# Autodesk Inventor assembly: slider
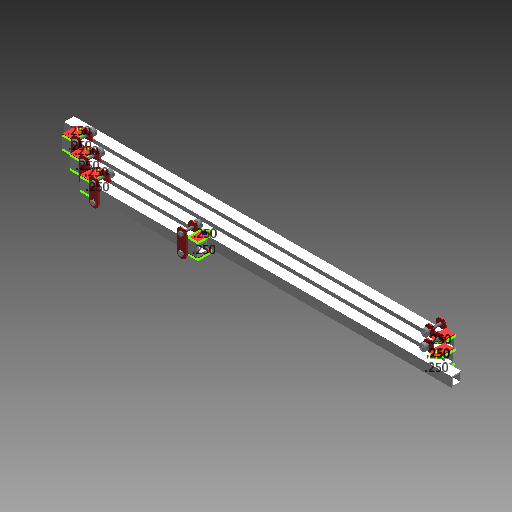
[picture p0: Inventor's stored thumbnail of the model, 512x512]
Saved by Autodesk Inventor 2019 (Build 230136000, 136)
## iProperties
Created: 2019-01-13
Part Number: slider
Document SubType Name: Assembly
Designer: lebraddock
Mass: 2872.54 g
Surface Area: 7390.42 cm^2
Volume: 1092.69 cm^3
Density: 2.62887 g/cm^3
Author: lebraddock
## Documents named in this file (9)
- C:\Users\lebraddock\Documents\CameronsRoboticsThings\2019 CAD\slider.iam
- C:\Users\lebraddock\Documents\CameronsRoboticsThings\2019 CAD\41inch 1x1 liftfirstbar.ipt
- C:\Users\lebraddock\Documents\CameronsRoboticsThings\2019 CAD\linear_slide_piece2_v2.ipt
- C:\Users\lebraddock\Documents\CameronsRoboticsThings\2019 CAD\linearSlide_piece1_v2.ipt
- C:\Users\lebraddock\Documents\CameronsRoboticsThings\2019 CAD\1x1 plate spacer.ipt
- C:\Users\lebraddock\Documents\CameronsRoboticsThings\2019 CAD\spacerslide.ipt
- C:\Users\lebraddock\Documents\CameronsRoboticsThings\2019 CAD\93306A555_ALUMINUM HEX HEAD CAP SCREW.ipt
- C:\Users\lebraddock\Documents\CameronsRoboticsThings\2019 CAD\60355K440_BALL BEARING.ipt
- C:\Users\lebraddock\Documents\CameronsRoboticsThings\2019 CAD\12sliderbar.ipt
## Components (70 placed, 8 different names)
1. 41inch 1x1 liftfirstbar:1 — Mate:1, Flush:1, Flush:2, Mate:2, Flush:3, Flush:4, Mate:3, Flush:5, Flush:6, Mate:4, Flush:7, Flush:8, Mate:5, Flush:9, Tangent:1, Mate:6, Flush:10, Tangent:2, Tangent:5, Tangent:7
2. linear_slide_piece2_v2:1 — Mate:6, Flush:10, Tangent:2, Mate:27, Mate:29
3. linearSlide_piece1_v2:1 — Mate:4, Flush:7, Flush:8, Mate:14
4. linear_slide_piece2_v2:2 — Mate:5, Flush:9, Tangent:1, Mate:19, Mate:20, Mate:21, Mate:22
5. linearSlide_piece1_v2:2 — Mate:1, Flush:1, Flush:2, Insert:2
6. 1x1 plate spacer:1 — Mate:3, Flush:5, Flush:6
7. 1x1 plate spacer:2 — Mate:2, Flush:3, Flush:4
8. spacerslide:2 — Mate:14, Insert:2, Tangent:6
9. 93306A555_ALUMINUM HEX HEAD CAP SCREW:1 — Mate:19, Mate:20, Mate:30
10. 93306A555_ALUMINUM HEX HEAD CAP SCREW:2 — Mate:21, Mate:22, Mate:28
11. 60355K440_BALL BEARING:1 — Mate:29, Mate:30, Tangent:8
12. 60355K440_BALL BEARING:2 — Mate:27, Mate:28
13. 12sliderbar:1 — Mate:99, Flush:53, Flush:54, Flush:55, Flush:56, Mate:101, Flush:57, Flush:58, Flush:59, Flush:60, Mate:103, Flush:61, Mate:104, Flush:62, Tangent:21, Tangent:22, Mate:105, Flush:63, Flush:64, Mate:106, Flush:65, Flush:66, Flush:68, Flush:69, Flush:70, Mate:110, Flush:71, Tangent:24, Mate:111, Flush:72, Tangent:25
14. 41inch 1x1 liftfirstbar:2 — Tangent:6, Tangent:8, Mate:68, Flush:31, Flush:32, Flush:33, Flush:34, Flush:35, Flush:36, Flush:37, Flush:38, Mate:70, Flush:39, Flush:40, Mate:72, Flush:41, Tangent:11, Mate:73, Flush:42, Tangent:17, Tangent:19
15. linear_slide_piece2_v2:3
16. linearSlide_piece1_v2:3
17. linear_slide_piece2_v2:4
18. linearSlide_piece1_v2:4
19. 1x1 plate spacer:3
20. 1x1 plate spacer:4
21. spacerslide:3 — Tangent:5
22. 93306A555_ALUMINUM HEX HEAD CAP SCREW:3
23. 93306A555_ALUMINUM HEX HEAD CAP SCREW:4
24. 60355K440_BALL BEARING:3 — Tangent:7
25. 60355K440_BALL BEARING:4
26. linear_slide_piece2_v2:7 — Mate:73, Flush:42
27. linearSlide_piece1_v2:7 — Mate:69, Flush:32, Flush:33, Flush:36, Mate:89
28. linear_slide_piece2_v2:8 — Mate:72, Flush:41
29. linearSlide_piece1_v2:8 — Mate:71, Flush:39, Flush:40, Tangent:15
30. 1x1 plate spacer:7 — Mate:68, Flush:31, Mate:69, Flush:34, Flush:35
31. 1x1 plate spacer:8 — Flush:37, Flush:38, Mate:70, Mate:71
32. 93306A555_ALUMINUM HEX HEAD CAP SCREW:7 — Tangent:11
33. 93306A555_ALUMINUM HEX HEAD CAP SCREW:8
34. 60355K440_BALL BEARING:7 — Tangent:16
35. 60355K440_BALL BEARING:8
36. 41inch 1x1 liftfirstbar:3 — Tangent:16, Tangent:18, Tangent:31, Tangent:32, Tangent:33, Tangent:34
37. linear_slide_piece2_v2:9
38. linearSlide_piece1_v2:9 — Mate:88
39. linear_slide_piece2_v2:10
40. linearSlide_piece1_v2:10 — Tangent:14
41. 1x1 plate spacer:9
42. 1x1 plate spacer:10
43. 93306A555_ALUMINUM HEX HEAD CAP SCREW:9
44. 93306A555_ALUMINUM HEX HEAD CAP SCREW:10
45. 60355K440_BALL BEARING:9 — Tangent:17
46. 60355K440_BALL BEARING:10
47. spacerslide:4 — Mate:89, Tangent:15, Tangent:18
48. spacerslide:5 — Mate:88, Tangent:14, Tangent:19
49. linear_slide_piece2_v2:11 — Mate:104, Flush:62, Tangent:22
50. linearSlide_piece1_v2:11 — Mate:102, Flush:59, Flush:60
51. linear_slide_piece2_v2:12 — Mate:103, Flush:61
52. linearSlide_piece1_v2:12 — Mate:100, Flush:55, Flush:56
53. 1x1 plate spacer:11 — Mate:101, Flush:57, Flush:58, Mate:102
54. 1x1 plate spacer:12 — Mate:99, Flush:53, Flush:54, Mate:100
55. 93306A555_ALUMINUM HEX HEAD CAP SCREW:11 — Tangent:21
56. 93306A555_ALUMINUM HEX HEAD CAP SCREW:12
57. 60355K440_BALL BEARING:11 — Tangent:31
58. 60355K440_BALL BEARING:12
59. spacerslide:6 — Tangent:33
60. linear_slide_piece2_v2:13 — Mate:110, Flush:71, Tangent:24, Mate:112, Mate:113
61. linearSlide_piece1_v2:13 — Mate:107, Flush:67, Flush:68, Mate:109
62. linear_slide_piece2_v2:14 — Mate:111, Flush:72, Tangent:25, Tangent:26, Mate:114, Tangent:29, Mate:115
63. linearSlide_piece1_v2:14 — Mate:108, Flush:69, Flush:70, Tangent:23
64. 1x1 plate spacer:13 — Mate:105, Flush:63, Flush:64, Mate:107, Flush:67
65. 1x1 plate spacer:14 — Mate:106, Flush:65, Flush:66, Mate:108
66. 60355K440_BALL BEARING:13 — Mate:115, Tangent:30
67. 60355K440_BALL BEARING:14 — Mate:114, Tangent:28, Tangent:32
68. spacerslide:7 — Mate:109, Tangent:23, Tangent:34
69. 93306A555_ALUMINUM HEX HEAD CAP SCREW:13 — Mate:112, Tangent:26, Tangent:28
70. 93306A555_ALUMINUM HEX HEAD CAP SCREW:14 — Mate:113, Tangent:29, Tangent:30
## Relationships (181: Mate 86, Flush 62, Tangent 31, Insert 2)
- Mate:1 (3.175 mm): 41inch 1x1 liftfirstbar:1 ↔ linearSlide_piece1_v2:2
- Flush:1: 41inch 1x1 liftfirstbar:1 ↔ linearSlide_piece1_v2:2
- Flush:2: 41inch 1x1 liftfirstbar:1 ↔ linearSlide_piece1_v2:2
- Mate:2: 41inch 1x1 liftfirstbar:1 ↔ 1x1 plate spacer:2
- Flush:3: 41inch 1x1 liftfirstbar:1 ↔ 1x1 plate spacer:2
- Flush:4: 41inch 1x1 liftfirstbar:1 ↔ 1x1 plate spacer:2
- Mate:3: 41inch 1x1 liftfirstbar:1 ↔ 1x1 plate spacer:1
- Flush:5: 41inch 1x1 liftfirstbar:1 ↔ 1x1 plate spacer:1
- Flush:6: 41inch 1x1 liftfirstbar:1 ↔ 1x1 plate spacer:1
- Mate:4 (3.175 mm): 41inch 1x1 liftfirstbar:1 ↔ linearSlide_piece1_v2:1
- Flush:7: 41inch 1x1 liftfirstbar:1 ↔ linearSlide_piece1_v2:1
- Flush:8: 41inch 1x1 liftfirstbar:1 ↔ linearSlide_piece1_v2:1
- Mate:5: 41inch 1x1 liftfirstbar:1 ↔ linear_slide_piece2_v2:2
- Flush:9 (25.4 mm): 41inch 1x1 liftfirstbar:1 ↔ linear_slide_piece2_v2:2
- Tangent:1 (6.35 mm): 41inch 1x1 liftfirstbar:1 ↔ linear_slide_piece2_v2:2
- Mate:6: 41inch 1x1 liftfirstbar:1 ↔ linear_slide_piece2_v2:1
- Flush:10 (25.4 mm): 41inch 1x1 liftfirstbar:1 ↔ linear_slide_piece2_v2:1
- Tangent:2 (6.35 mm): 41inch 1x1 liftfirstbar:1 ↔ linear_slide_piece2_v2:1
- Mate:14: linearSlide_piece1_v2:1 ↔ spacerslide:2
- Insert:2: linearSlide_piece1_v2:2 ↔ spacerslide:2
- Mate:19: linear_slide_piece2_v2:2 ↔ 93306A555_ALUMINUM HEX HEAD CAP SCREW:1
- Mate:20: linear_slide_piece2_v2:2 ↔ 93306A555_ALUMINUM HEX HEAD CAP SCREW:1
- Mate:21: linear_slide_piece2_v2:2 ↔ 93306A555_ALUMINUM HEX HEAD CAP SCREW:2
- Mate:22: linear_slide_piece2_v2:2 ↔ 93306A555_ALUMINUM HEX HEAD CAP SCREW:2
- Mate:27 (7.112 mm): linear_slide_piece2_v2:1 ↔ 60355K440_BALL BEARING:2
- Mate:28: 93306A555_ALUMINUM HEX HEAD CAP SCREW:2 ↔ 60355K440_BALL BEARING:2
- Mate:29 (7.112 mm): linear_slide_piece2_v2:1 ↔ 60355K440_BALL BEARING:1
- Mate:30: 93306A555_ALUMINUM HEX HEAD CAP SCREW:1 ↔ 60355K440_BALL BEARING:1
- [Mate] (3.175 mm): 41inch 1x1 liftfirstbar:2 ↔ linearSlide_piece1_v2:4
- [Flush]: 41inch 1x1 liftfirstbar:2 ↔ linearSlide_piece1_v2:4
- [Flush]: 41inch 1x1 liftfirstbar:2 ↔ linearSlide_piece1_v2:4
- [Mate]: 41inch 1x1 liftfirstbar:2 ↔ 1x1 plate spacer:4
- [Flush]: 41inch 1x1 liftfirstbar:2 ↔ 1x1 plate spacer:4
- [Flush]: 41inch 1x1 liftfirstbar:2 ↔ 1x1 plate spacer:4
- [Mate]: 41inch 1x1 liftfirstbar:2 ↔ 1x1 plate spacer:3
- [Flush]: 41inch 1x1 liftfirstbar:2 ↔ 1x1 plate spacer:3
- [Flush]: 41inch 1x1 liftfirstbar:2 ↔ 1x1 plate spacer:3
- [Mate] (3.175 mm): 41inch 1x1 liftfirstbar:2 ↔ linearSlide_piece1_v2:3
- [Flush]: 41inch 1x1 liftfirstbar:2 ↔ linearSlide_piece1_v2:3
- [Flush]: 41inch 1x1 liftfirstbar:2 ↔ linearSlide_piece1_v2:3
- [Mate]: 41inch 1x1 liftfirstbar:2 ↔ linear_slide_piece2_v2:4
- [Flush] (25.4 mm): 41inch 1x1 liftfirstbar:2 ↔ linear_slide_piece2_v2:4
- [Tangent] (6.35 mm): 41inch 1x1 liftfirstbar:2 ↔ linear_slide_piece2_v2:4
- [Mate]: 41inch 1x1 liftfirstbar:2 ↔ linear_slide_piece2_v2:3
- [Flush] (25.4 mm): 41inch 1x1 liftfirstbar:2 ↔ linear_slide_piece2_v2:3
- [Tangent] (6.35 mm): 41inch 1x1 liftfirstbar:2 ↔ linear_slide_piece2_v2:3
- [Mate]: linearSlide_piece1_v2:3 ↔ spacerslide:3
- [Insert]: linearSlide_piece1_v2:4 ↔ spacerslide:3
- [Mate]: linear_slide_piece2_v2:4 ↔ 93306A555_ALUMINUM HEX HEAD CAP SCREW:3
- [Mate]: linear_slide_piece2_v2:4 ↔ 93306A555_ALUMINUM HEX HEAD CAP SCREW:3
- [Mate]: linear_slide_piece2_v2:4 ↔ 93306A555_ALUMINUM HEX HEAD CAP SCREW:4
- [Mate]: linear_slide_piece2_v2:4 ↔ 93306A555_ALUMINUM HEX HEAD CAP SCREW:4
- [Mate] (7.112 mm): linear_slide_piece2_v2:3 ↔ 60355K440_BALL BEARING:4
- [Mate]: 93306A555_ALUMINUM HEX HEAD CAP SCREW:4 ↔ 60355K440_BALL BEARING:4
- [Mate] (7.112 mm): linear_slide_piece2_v2:3 ↔ 60355K440_BALL BEARING:3
- [Mate]: 93306A555_ALUMINUM HEX HEAD CAP SCREW:3 ↔ 60355K440_BALL BEARING:3
- Tangent:5: 41inch 1x1 liftfirstbar:1 ↔ spacerslide:3
- Tangent:6: spacerslide:2 ↔ 41inch 1x1 liftfirstbar:2
- Tangent:7: 41inch 1x1 liftfirstbar:1 ↔ 60355K440_BALL BEARING:3
- Tangent:8: 60355K440_BALL BEARING:1 ↔ 41inch 1x1 liftfirstbar:2
- [Mate]: linear_slide_piece2_v2:8 ↔ 93306A555_ALUMINUM HEX HEAD CAP SCREW:7
- [Mate]: linear_slide_piece2_v2:8 ↔ 93306A555_ALUMINUM HEX HEAD CAP SCREW:7
- [Mate]: linear_slide_piece2_v2:8 ↔ 93306A555_ALUMINUM HEX HEAD CAP SCREW:8
- [Mate]: linear_slide_piece2_v2:8 ↔ 93306A555_ALUMINUM HEX HEAD CAP SCREW:8
- [Mate] (7.112 mm): linear_slide_piece2_v2:7 ↔ 60355K440_BALL BEARING:8
- [Mate]: 93306A555_ALUMINUM HEX HEAD CAP SCREW:8 ↔ 60355K440_BALL BEARING:8
- [Mate] (7.112 mm): linear_slide_piece2_v2:7 ↔ 60355K440_BALL BEARING:7
- [Mate]: 93306A555_ALUMINUM HEX HEAD CAP SCREW:7 ↔ 60355K440_BALL BEARING:7
- Mate:68: 41inch 1x1 liftfirstbar:2 ↔ 1x1 plate spacer:7
- Flush:31: 41inch 1x1 liftfirstbar:2 ↔ 1x1 plate spacer:7
- Mate:69: linearSlide_piece1_v2:7 ↔ 1x1 plate spacer:7
- Flush:32: 41inch 1x1 liftfirstbar:2 ↔ linearSlide_piece1_v2:7
- Flush:33: 41inch 1x1 liftfirstbar:2 ↔ linearSlide_piece1_v2:7
- Flush:34: 41inch 1x1 liftfirstbar:2 ↔ 1x1 plate spacer:7
- Flush:35: 41inch 1x1 liftfirstbar:2 ↔ 1x1 plate spacer:7
- Flush:36: 41inch 1x1 liftfirstbar:2 ↔ linearSlide_piece1_v2:7
- Flush:37: 41inch 1x1 liftfirstbar:2 ↔ 1x1 plate spacer:8
- Flush:38: 41inch 1x1 liftfirstbar:2 ↔ 1x1 plate spacer:8
- Mate:70: 41inch 1x1 liftfirstbar:2 ↔ 1x1 plate spacer:8
- Mate:71: linearSlide_piece1_v2:8 ↔ 1x1 plate spacer:8
- Flush:39: 41inch 1x1 liftfirstbar:2 ↔ linearSlide_piece1_v2:8
- Flush:40: 41inch 1x1 liftfirstbar:2 ↔ linearSlide_piece1_v2:8
- Mate:72: 41inch 1x1 liftfirstbar:2 ↔ linear_slide_piece2_v2:8
- Flush:41 (25.4 mm): 41inch 1x1 liftfirstbar:2 ↔ linear_slide_piece2_v2:8
- Tangent:11 (6.35 mm): 41inch 1x1 liftfirstbar:2 ↔ 93306A555_ALUMINUM HEX HEAD CAP SCREW:7
- Mate:73: 41inch 1x1 liftfirstbar:2 ↔ linear_slide_piece2_v2:7
- Flush:42 (25.4 mm): 41inch 1x1 liftfirstbar:2 ↔ linear_slide_piece2_v2:7
- [Mate] (3.175 mm): 41inch 1x1 liftfirstbar:3 ↔ linearSlide_piece1_v2:10
- [Flush]: 41inch 1x1 liftfirstbar:3 ↔ linearSlide_piece1_v2:10
- [Flush]: 41inch 1x1 liftfirstbar:3 ↔ linearSlide_piece1_v2:10
- [Mate]: 41inch 1x1 liftfirstbar:3 ↔ 1x1 plate spacer:10
- [Flush]: 41inch 1x1 liftfirstbar:3 ↔ 1x1 plate spacer:10
- [Flush]: 41inch 1x1 liftfirstbar:3 ↔ 1x1 plate spacer:10
- [Mate]: 41inch 1x1 liftfirstbar:3 ↔ 1x1 plate spacer:9
- [Flush]: 41inch 1x1 liftfirstbar:3 ↔ 1x1 plate spacer:9
- [Flush]: 41inch 1x1 liftfirstbar:3 ↔ 1x1 plate spacer:9
- [Mate] (3.175 mm): 41inch 1x1 liftfirstbar:3 ↔ linearSlide_piece1_v2:9
- [Flush]: 41inch 1x1 liftfirstbar:3 ↔ linearSlide_piece1_v2:9
- [Flush]: 41inch 1x1 liftfirstbar:3 ↔ linearSlide_piece1_v2:9
- [Mate]: 41inch 1x1 liftfirstbar:3 ↔ linear_slide_piece2_v2:10
- [Flush] (25.4 mm): 41inch 1x1 liftfirstbar:3 ↔ linear_slide_piece2_v2:10
- [Tangent] (6.35 mm): 41inch 1x1 liftfirstbar:3 ↔ linear_slide_piece2_v2:10
- [Mate]: 41inch 1x1 liftfirstbar:3 ↔ linear_slide_piece2_v2:9
- [Flush] (25.4 mm): 41inch 1x1 liftfirstbar:3 ↔ linear_slide_piece2_v2:9
- [Tangent] (6.35 mm): 41inch 1x1 liftfirstbar:3 ↔ linear_slide_piece2_v2:9
- [Mate]: linear_slide_piece2_v2:10 ↔ 93306A555_ALUMINUM HEX HEAD CAP SCREW:9
- [Mate]: linear_slide_piece2_v2:10 ↔ 93306A555_ALUMINUM HEX HEAD CAP SCREW:9
- [Mate]: linear_slide_piece2_v2:10 ↔ 93306A555_ALUMINUM HEX HEAD CAP SCREW:10
- [Mate]: linear_slide_piece2_v2:10 ↔ 93306A555_ALUMINUM HEX HEAD CAP SCREW:10
- [Mate] (7.112 mm): linear_slide_piece2_v2:9 ↔ 60355K440_BALL BEARING:10
- [Mate]: 93306A555_ALUMINUM HEX HEAD CAP SCREW:10 ↔ 60355K440_BALL BEARING:10
- [Mate] (7.112 mm): linear_slide_piece2_v2:9 ↔ 60355K440_BALL BEARING:9
- [Mate]: 93306A555_ALUMINUM HEX HEAD CAP SCREW:9 ↔ 60355K440_BALL BEARING:9
- Mate:88: linearSlide_piece1_v2:9 ↔ spacerslide:5
- Tangent:14: linearSlide_piece1_v2:10 ↔ spacerslide:5
- Mate:89: linearSlide_piece1_v2:7 ↔ spacerslide:4
- Tangent:15: linearSlide_piece1_v2:8 ↔ spacerslide:4
- Tangent:16: 60355K440_BALL BEARING:7 ↔ 41inch 1x1 liftfirstbar:3
- Tangent:17: 41inch 1x1 liftfirstbar:2 ↔ 60355K440_BALL BEARING:9
- Tangent:18: 41inch 1x1 liftfirstbar:3 ↔ spacerslide:4
- Tangent:19: 41inch 1x1 liftfirstbar:2 ↔ spacerslide:5
- [Mate]: linear_slide_piece2_v2:12 ↔ 93306A555_ALUMINUM HEX HEAD CAP SCREW:11
- [Mate]: linear_slide_piece2_v2:12 ↔ 93306A555_ALUMINUM HEX HEAD CAP SCREW:11
- [Mate]: linear_slide_piece2_v2:12 ↔ 93306A555_ALUMINUM HEX HEAD CAP SCREW:12
- [Mate]: linear_slide_piece2_v2:12 ↔ 93306A555_ALUMINUM HEX HEAD CAP SCREW:12
- [Mate] (7.112 mm): linear_slide_piece2_v2:11 ↔ 60355K440_BALL BEARING:12
- [Mate]: 93306A555_ALUMINUM HEX HEAD CAP SCREW:12 ↔ 60355K440_BALL BEARING:12
- [Mate] (7.112 mm): linear_slide_piece2_v2:11 ↔ 60355K440_BALL BEARING:11
- [Mate]: 93306A555_ALUMINUM HEX HEAD CAP SCREW:11 ↔ 60355K440_BALL BEARING:11
- [Mate]: linearSlide_piece1_v2:11 ↔ spacerslide:6
- [Tangent]: linearSlide_piece1_v2:12 ↔ spacerslide:6
- Mate:99: 12sliderbar:1 ↔ 1x1 plate spacer:12
- Flush:53: 12sliderbar:1 ↔ 1x1 plate spacer:12
- Flush:54: 12sliderbar:1 ↔ 1x1 plate spacer:12
- Mate:100: linearSlide_piece1_v2:12 ↔ 1x1 plate spacer:12
- Flush:55: 12sliderbar:1 ↔ linearSlide_piece1_v2:12
- Flush:56: 12sliderbar:1 ↔ linearSlide_piece1_v2:12
- Mate:101: 12sliderbar:1 ↔ 1x1 plate spacer:11
- Flush:57: 12sliderbar:1 ↔ 1x1 plate spacer:11
- Flush:58: 12sliderbar:1 ↔ 1x1 plate spacer:11
- Mate:102: linearSlide_piece1_v2:11 ↔ 1x1 plate spacer:11
- Flush:59: 12sliderbar:1 ↔ linearSlide_piece1_v2:11
- Flush:60: 12sliderbar:1 ↔ linearSlide_piece1_v2:11
- Mate:103: 12sliderbar:1 ↔ linear_slide_piece2_v2:12
- Flush:61 (25.4 mm): 12sliderbar:1 ↔ linear_slide_piece2_v2:12
- Mate:104: 12sliderbar:1 ↔ linear_slide_piece2_v2:11
- Flush:62 (25.4 mm): 12sliderbar:1 ↔ linear_slide_piece2_v2:11
- Tangent:21 (6.35 mm): 12sliderbar:1 ↔ 93306A555_ALUMINUM HEX HEAD CAP SCREW:11
- Tangent:22 (6.35 mm): 12sliderbar:1 ↔ linear_slide_piece2_v2:11
- Mate:105: 12sliderbar:1 ↔ 1x1 plate spacer:13
- Flush:63: 12sliderbar:1 ↔ 1x1 plate spacer:13
- Flush:64: 12sliderbar:1 ↔ 1x1 plate spacer:13
- Mate:106: 12sliderbar:1 ↔ 1x1 plate spacer:14
- Flush:65: 12sliderbar:1 ↔ 1x1 plate spacer:14
- Flush:66: 12sliderbar:1 ↔ 1x1 plate spacer:14
- Mate:107: linearSlide_piece1_v2:13 ↔ 1x1 plate spacer:13
- Flush:67: linearSlide_piece1_v2:13 ↔ 1x1 plate spacer:13
- Flush:68: 12sliderbar:1 ↔ linearSlide_piece1_v2:13
- Mate:108: linearSlide_piece1_v2:14 ↔ 1x1 plate spacer:14
- Flush:69: 12sliderbar:1 ↔ linearSlide_piece1_v2:14
- Flush:70: 12sliderbar:1 ↔ linearSlide_piece1_v2:14
- Mate:109: linearSlide_piece1_v2:13 ↔ spacerslide:7
- Tangent:23: linearSlide_piece1_v2:14 ↔ spacerslide:7
- Mate:110: 12sliderbar:1 ↔ linear_slide_piece2_v2:13
- Flush:71 (25.4 mm): 12sliderbar:1 ↔ linear_slide_piece2_v2:13
- Tangent:24 (6.35 mm): 12sliderbar:1 ↔ linear_slide_piece2_v2:13
- Mate:111: 12sliderbar:1 ↔ linear_slide_piece2_v2:14
- Flush:72 (25.4 mm): 12sliderbar:1 ↔ linear_slide_piece2_v2:14
- Tangent:25 (6.35 mm): 12sliderbar:1 ↔ linear_slide_piece2_v2:14
- Mate:112: linear_slide_piece2_v2:13 ↔ 93306A555_ALUMINUM HEX HEAD CAP SCREW:13
- Mate:113: linear_slide_piece2_v2:13 ↔ 93306A555_ALUMINUM HEX HEAD CAP SCREW:14
- Tangent:26: linear_slide_piece2_v2:14 ↔ 93306A555_ALUMINUM HEX HEAD CAP SCREW:13
- Mate:114 (7.112 mm): linear_slide_piece2_v2:14 ↔ 60355K440_BALL BEARING:14
- Tangent:28: 60355K440_BALL BEARING:14 ↔ 93306A555_ALUMINUM HEX HEAD CAP SCREW:13
- Tangent:29: linear_slide_piece2_v2:14 ↔ 93306A555_ALUMINUM HEX HEAD CAP SCREW:14
- Mate:115 (7.112 mm): linear_slide_piece2_v2:14 ↔ 60355K440_BALL BEARING:13
- Tangent:30: 60355K440_BALL BEARING:13 ↔ 93306A555_ALUMINUM HEX HEAD CAP SCREW:14
- Tangent:31: 41inch 1x1 liftfirstbar:3 ↔ 60355K440_BALL BEARING:11
- Tangent:32: 41inch 1x1 liftfirstbar:3 ↔ 60355K440_BALL BEARING:14
- Tangent:33: 41inch 1x1 liftfirstbar:3 ↔ spacerslide:6
- Tangent:34: 41inch 1x1 liftfirstbar:3 ↔ spacerslide:7
## Named parameters: d116_d3 = 0 mm, d117_d4 = 0 mm, d118_d5 = 0 mm, d119_d6 = 0 mm, d120_d7 = 0 mm, d121_d8 = 0 mm, d122_d9 = 3.175 mm, d123_d10 = 0 mm, d124_d11 = 0 mm, d125_d12 = 0 mm, d126_d13 = 25.4 mm, d127_d38 = 0 mm, d128_d39 = 0 mm, d129_d44 = 0 mm, d130_d45 = 0 mm, d131_d46 = 0 mm, d132_d14 = 6.35 mm, d133_d15 = 0 mm, d134_d16 = 25.4 mm, d135_d17 = 6.35 mm, d136_d0 = 3.175 mm, d137_d1 = 0 mm, d138_d2 = 0 mm, d139_d47 = 0 mm, d140_d52 = 7.112 mm, d141_d53 = 0 mm, d142_d54 = 7.112 mm, d143_d55 = 0 mm, d174_d44 = 0 mm, d175_d45 = 0 mm, d176_d46 = 0 mm, d177_d47 = 0 mm, d178_d52 = 7.112 mm, d179_d53 = 0 mm, d180_d54 = 7.112 mm, d181_d55 = 0 mm, d201_d116_d3 = 0 mm, d202_d117_d4 = 0 mm, d203_d118_d5 = 0 mm, d204_d119_d6 = 0 mm, d205_d120_d7 = 0 mm, d206_d121_d8 = 0 mm, d207_d122_d9 = 3.175 mm, d208_d123_d10 = 0 mm, d209_d124_d11 = 0 mm, d210_d125_d12 = 0 mm, d211_d126_d13 = 25.4 mm, d212_d129_d44 = 0 mm, d213_d130_d45 = 0 mm, d214_d131_d46 = 0 mm, d215_d132_d14 = 6.35 mm, d216_d133_d15 = 0 mm, d217_d134_d16 = 25.4 mm, d218_d135_d17 = 6.35 mm, d219_d136_d0 = 3.175 mm, d220_d137_d1 = 0 mm, d221_d138_d2 = 0 mm, d222_d139_d47 = 0 mm, d223_d140_d52 = 7.112 mm, d224_d141_d53 = 0 mm, d225_d142_d54 = 7.112 mm, d226_d143_d55 = 0 mm, d235_d212_d129_d44 = 0 mm, d236_d213_d130_d45 = 0 mm, d237_d214_d131_d46 = 0 mm, d238_d222_d139_d47 = 0 mm, d239_d223_d140_d52 = 7.112 mm, d240_d224_d141_d53 = 0 mm, d241_d225_d142_d54 = 7.112 mm, d242_d226_d143_d55 = 0 mm, d243_d227 = 0 mm, d244_d228 = 0 mm
